# Autodesk Inventor assembly: new wind guide4 - shorter
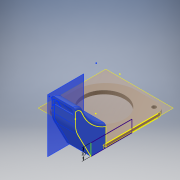
[picture p0: Inventor's stored thumbnail of the model, 180x180]
Saved by Autodesk Inventor 2016 (Build 200138000, 138)
## iProperties
Created: 2016-01-18
Part Number: new wind guide4 - shorter
Document SubType Name: Assembly
Designer: Erwin Ried
Author: Erwin Ried
## Documents named in this file (4)
- D:\OneDrive\RepRap\Parts\New\new wind\new wind guide4 - shorter.iam
- D:\OneDrive\RepRap\Parts\New\new wind\base.ipt
- D:\OneDrive\RepRap\Parts\New\new wind\guide.ipt
- D:\OneDrive\RepRap\Parts\New\new wind\sensor.ipt
## Components (3 placed, 3 different names)
1. base:1 — Flush:1, Flush:2
2. guide:1
3. sensor:1 — Flush:1, Flush:2
## Relationships (2: Flush 2)
- Flush:1: base:1 ↔ sensor:1
- Flush:2: base:1 ↔ sensor:1
